# Autodesk Inventor assembly: enormous-gear
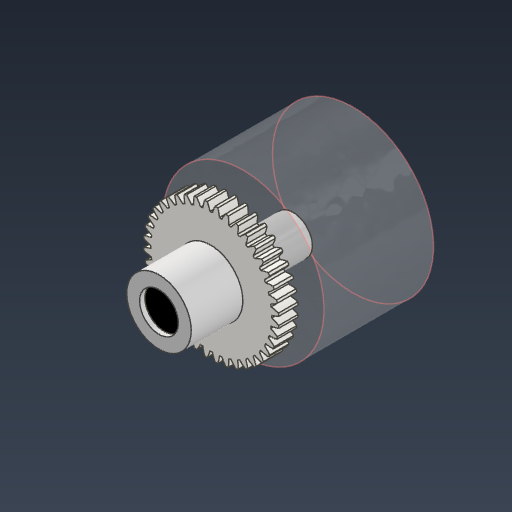
[picture p0: Inventor's stored thumbnail of the model, 512x512]
Saved by Autodesk Inventor 2023 (Build 270158000, 158)
## iProperties
Created: 2025-04-01
Part Number: enormous-gear
Document SubType Name: Assembly
Designer: szymo
Author: szymo
## Documents named in this file (4)
- D:\tech\robotyka\robots\evangelion\inventor-project\enormous-gear.iam
- D:\tech\robotyka\robots\evangelion\inventor-project\Gears\Design Accelerator\Przekładnia walcowa24.ipt
- D:\tech\robotyka\robots\evangelion\inventor-project\Lozysko HK0608.ipt
- D:\tech\robotyka\robots\evangelion\inventor-project\oponka-dziurawa-prototyp\wheel.ipt
## Components (3 placed, 3 different names)
1. Przekładnia walcowa2:1 — Mate:1, Mate:2, Mate:3, Mate:4
2. Lozysko HK0608:1 — Mate:1, Mate:2
3. wheel:1 — Mate:3, Mate:4
## Relationships (4: Mate 4)
- Mate:1: Przekładnia walcowa2:1 ↔ Lozysko HK0608:1
- Mate:2 (0.1 mm): Przekładnia walcowa2:1 ↔ Lozysko HK0608:1
- Mate:3: Przekładnia walcowa2:1 ↔ wheel:1
- Mate:4 (2 mm): Przekładnia walcowa2:1 ↔ wheel:1
